# Autodesk Inventor assembly: DribblerUnit
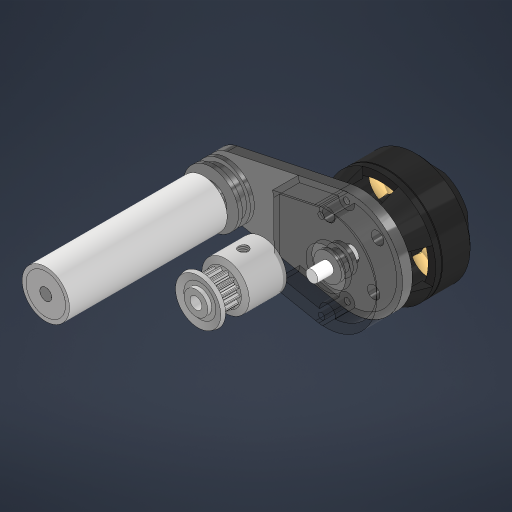
[picture p0: Inventor's stored thumbnail of the model, 512x512]
Saved by Autodesk Inventor 2024.2 (Build 282272000, 272)
## iProperties
Created: 2023-12-22
Part Number: DribblerUnit
Document SubType Name: Assembly
Designer: Hanaoka
Author: Hanaoka
## Documents named in this file (11)
- G:\共有ドライブ\reRo\05_個人\hanaoka\inventor\DribblerUnit.iam
- G:\共有ドライブ\reRo\05_個人\hanaoka\inventor\SilliconeTube_Dribbler.ipt
- G:\共有ドライブ\reRo\05_個人\hanaoka\inventor\C2822_BLDC\C2822_BLDC.ipt
- G:\共有ドライブ\reRo\05_個人\hanaoka\inventor\Dribler_main.ipt
- G:\共有ドライブ\reRo\05_個人\hanaoka\inventor\Misumi\Bearing_C-FL673ZZ\Bearing_C-FL673ZZ.ipt
- G:\共有ドライブ\reRo\05_個人\hanaoka\inventor\Shaft_3x50.ipt
- G:\共有ドライブ\reRo\05_個人\hanaoka\inventor\Pulley_MotorSide.ipt
- G:\共有ドライブ\reRo\05_個人\hanaoka\inventor\Pulley_OutSide.ipt
- G:\共有ドライブ\reRo\05_個人\hanaoka\inventor\MotorCover.ipt
- G:\共有ドライブ\reRo\05_個人\hanaoka\inventor\加工指示\SilliconeTube_Mount.ipt
- G:\共有ドライブ\reRo\05_個人\hanaoka\inventor\HTPB14S2M040-K-P3\HTPB14S2M040-K-P3.iam
## Components (10 placed, 10 different names)
1. SilliconeTube_Dribbler:1 — 挿入:5, メイト:1
2. C2822_BLDC:1 — フラッシュ:1, 挿入:3
3. Dribler_main:1 — フラッシュ:1, 挿入:1, フラッシュ:2, フラッシュ:3
4. Bearing_C-FL673ZZ:1 — 挿入:1, 挿入:2, 挿入:4
5. Shaft_3x50:1 — 挿入:2, メイト:1, フラッシュ:4
6. Pulley_MotorSide:1 — 挿入:3
7. Pulley_OutSide:1 — 挿入:4
8. MotorCover:1 — フラッシュ:2, フラッシュ:3
9. SilliconeTube_Mount:1 — 挿入:5, フラッシュ:4
10. HTPB14S2M040-K-P3:1 [sub-assembly]
## Relationships (10: Insert 5, Flush 4, Mate 1)
- フラッシュ:1 [Flush]: C2822_BLDC:1 ↔ Dribler_main:1
- 挿入:1 [Insert]: Dribler_main:1 ↔ Bearing_C-FL673ZZ:1
- 挿入:2 [Insert]: Bearing_C-FL673ZZ:1 ↔ Shaft_3x50:1
- 挿入:3 [Insert] (4 mm): C2822_BLDC:1 ↔ Pulley_MotorSide:1
- フラッシュ:2 [Flush]: Dribler_main:1 ↔ MotorCover:1
- フラッシュ:3 [Flush]: Dribler_main:1 ↔ MotorCover:1
- 挿入:4 [Insert] (4 mm): Bearing_C-FL673ZZ:1 ↔ Pulley_OutSide:1
- 挿入:5 [Insert]: SilliconeTube_Dribbler:1 ↔ SilliconeTube_Mount:1
- メイト:1 [Mate]: SilliconeTube_Dribbler:1 ↔ Shaft_3x50:1
- フラッシュ:4 [Flush]: Shaft_3x50:1 ↔ SilliconeTube_Mount:1
